# Autodesk Inventor assembly: DriveTrainMotor+MountC
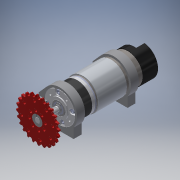
[picture p0: Inventor's stored thumbnail of the model, 180x180]
Saved by Autodesk Inventor 2018 (Build 220112000, 112)
## iProperties
Created: 2017-11-14
Part Number: DriveTrainMotor+MountC
Document SubType Name: Assembly
Designer: ball
Author: ball
## Documents named in this file (5)
- C:\FTC\FTC8863CAD\2017Robot\DriveTrainMotor+MountC.iam
- C:\FTC\FTC8863CAD\Andymark\am-3461a+NeveRest+Orbital+3.7+REV2.ipt
- C:\FTC\FTC8863CAD\Actobotics\615 parts\615106.ipt
- C:\FTC\FTC8863CAD\Actobotics\545 parts\545618 assembly.ipt
- C:\FTC\FTC8863CAD\Actobotics\555 parts\555116.ipt
## Components (5 placed, 4 different names)
1. am-3461a+NeveRest+Orbital+3.7+REV2:1 — Mate:16, Flush:1, Flush:2, Mate:17, Mate:18, Flush:4, Flush:5
2. 615106:2 — Mate:13, Mate:14, Mate:15
3. 545618 assembly:2 — Mate:13, Mate:14, Mate:15, Mate:16, Flush:1, Flush:2
4. 555116:1 — Mate:17, Flush:3, Flush:5
5. 555116:2 — Mate:18, Flush:3, Flush:4
## Relationships (11: Mate 6, Flush 5)
- Mate:13: 615106:2 ↔ 545618 assembly:2
- Mate:14: 615106:2 ↔ 545618 assembly:2
- Mate:15: 615106:2 ↔ 545618 assembly:2
- Mate:16: am-3461a+NeveRest+Orbital+3.7+REV2:1 ↔ 545618 assembly:2
- Flush:1: am-3461a+NeveRest+Orbital+3.7+REV2:1 ↔ 545618 assembly:2
- Flush:2: am-3461a+NeveRest+Orbital+3.7+REV2:1 ↔ 545618 assembly:2
- Mate:17: am-3461a+NeveRest+Orbital+3.7+REV2:1 ↔ 555116:1
- Mate:18: am-3461a+NeveRest+Orbital+3.7+REV2:1 ↔ 555116:2
- Flush:3: 555116:1 ↔ 555116:2
- Flush:4: am-3461a+NeveRest+Orbital+3.7+REV2:1 ↔ 555116:2
- Flush:5 (25.4 mm): am-3461a+NeveRest+Orbital+3.7+REV2:1 ↔ 555116:1
